# Autodesk Inventor assembly: B30041_MIR
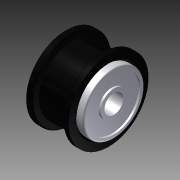
[picture p0: Inventor's stored thumbnail of the model, 180x180]
Saved by Autodesk Inventor 2014 (Build 180170000, 170)
## iProperties
Created: 2012-01-24
Part Number: B30041_MIR
Catalog Web Link: varies
Description: Smooth Idler Assembly
Vendor: custom
Document SubType Name: Assembly
Designer: Edward
Stock Number: B30041_ASM
Mass: 2.21849 g
Surface Area: 41.2914 cm^2
Volume: 1.85724 cm^3
Density: 1.19451 g/cm^3
Author: ERF
## Documents named in this file (4)
- C:\Users\Edward\Desktop\Shapeoko_v2.0\B30041_MIR.iam
- C:\Users\Edward\Desktop\Shapeoko_v2.0\B18026_MIR.ipt
- C:\Users\Edward\Desktop\Shapeoko_v2.0\BEARING_5_16_5_MIR.ipt
- C:\Users\Edward\Desktop\Shapeoko_v2.0\B17023_MIR.ipt
## Components (4 placed, 3 different names)
1. B18026_MIR:1 — Insert:3, Insert:2
2. BEARING_5_16_5_MIR:1 — Insert:3
3. BEARING_5_16_5_MIR:2 — Insert:2, Insert:1
4. B17023_MIR:1 — Insert:1
## Relationships (3: Insert 3)
- Insert:3: B18026_MIR:1 ↔ BEARING_5_16_5_MIR:1
- Insert:2: B18026_MIR:1 ↔ BEARING_5_16_5_MIR:2
- Insert:1: BEARING_5_16_5_MIR:2 ↔ B17023_MIR:1
